# Autodesk Inventor assembly: GameBoy
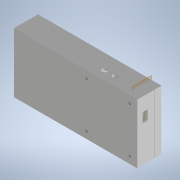
[picture p0: Inventor's stored thumbnail of the model, 180x180]
Saved by Autodesk Inventor 2022 (Build 260153000, 153)
## iProperties
Created: 2023-09-02
Part Number: GameBoy
Document SubType Name: Assembly
Designer: Petr Černý
Author: Petr Černý
## Documents named in this file (7)
- C:\Projekty\GameBoy\3D Model\GameBoy.iam
- C:\Projekty\GameBoy\3D Model\LowerHalf.ipt
- C:\Projekty\GameBoy\3D Model\Upper_Half.ipt
- C:\Projekty\GameBoy\3D Model\GameBoy_PCB.iam
- C:\Projekty\GameBoy\3D Model\Nokia5110.iam
- C:\Projekty\GameBoy\3D Model\Tactile_Push_Button.ipt
- C:\Projekty\GameBoy\3D Model\3x AAA battery holder_update.iam
## Components (10 placed, 6 different names)
1. LowerHalf:1 — Mate:1, Mate:2, Mate:3, Flush:9, Flush:10, Mate:12, Mate:13
2. Upper_Half:1 — Mate:4, Mate:5, Mate:6, Mate:7, Flush:2, Flush:3, Mate:8, Flush:4, Flush:5, Mate:9, Flush:6, Flush:7, Mate:10, Mate:11, Flush:8, Flush:9, Flush:10, Flush:11, Mate:14, Flush:12, Flush:13
3. GameBoy_PCB:1 [sub-assembly] — Mate:1, Mate:2, Mate:3
4. Nokia5110:1 [sub-assembly] — Mate:4, Mate:5, Mate:6
5. Tactile_Push_Button:1 — Mate:7, Flush:2, Flush:3
6. Tactile_Push_Button:2 — Mate:8, Flush:4, Flush:5
7. Tactile_Push_Button:3 — Mate:10, Mate:11, Flush:8
8. Tactile_Push_Button:4 — Mate:9, Flush:6, Flush:7
9. 3x AAA battery holder_update:1 [sub-assembly] — Mate:12, Mate:13
10. Tactile_Push_Button:5 — Mate:14, Flush:12, Flush:13
## Relationships (26: Mate 14, Flush 12)
- Mate:1: LowerHalf:1 ↔ GameBoy_PCB:1
- Mate:2 (1 mm): LowerHalf:1 ↔ GameBoy_PCB:1
- Mate:3 (1.5 mm): LowerHalf:1 ↔ GameBoy_PCB:1
- Mate:4: Upper_Half:1 ↔ Nokia5110:1
- Mate:5: Upper_Half:1 ↔ Nokia5110:1
- Mate:6: Upper_Half:1 ↔ Nokia5110:1
- Mate:7: Upper_Half:1 ↔ Tactile_Push_Button:1
- Flush:2 (10.25 mm): Upper_Half:1 ↔ Tactile_Push_Button:1
- Flush:3 (24.5 mm): Upper_Half:1 ↔ Tactile_Push_Button:1
- Mate:8: Upper_Half:1 ↔ Tactile_Push_Button:2
- Flush:4 (24.5 mm): Upper_Half:1 ↔ Tactile_Push_Button:2
- Flush:5 (10 mm): Upper_Half:1 ↔ Tactile_Push_Button:2
- Mate:9: Upper_Half:1 ↔ Tactile_Push_Button:4
- Flush:6 (10 mm): Upper_Half:1 ↔ Tactile_Push_Button:4
- Flush:7 (24.5 mm): Upper_Half:1 ↔ Tactile_Push_Button:4
- Mate:10: Upper_Half:1 ↔ Tactile_Push_Button:3
- Mate:11 (-30.5 mm): Upper_Half:1 ↔ Tactile_Push_Button:3
- Flush:8 (39 mm): Upper_Half:1 ↔ Tactile_Push_Button:3
- Flush:9: LowerHalf:1 ↔ Upper_Half:1
- Flush:10: LowerHalf:1 ↔ Upper_Half:1
- Flush:11 (-10 mm): Upper_Half:1
- Mate:12: LowerHalf:1 ↔ 3x AAA battery holder_update:1
- Mate:13: LowerHalf:1 ↔ 3x AAA battery holder_update:1
- Mate:14: Upper_Half:1 ↔ Tactile_Push_Button:5
- Flush:12 (51.2 mm): Upper_Half:1 ↔ Tactile_Push_Button:5
- Flush:13 (10 mm): Upper_Half:1 ↔ Tactile_Push_Button:5
